# Autodesk Inventor assembly: assembly
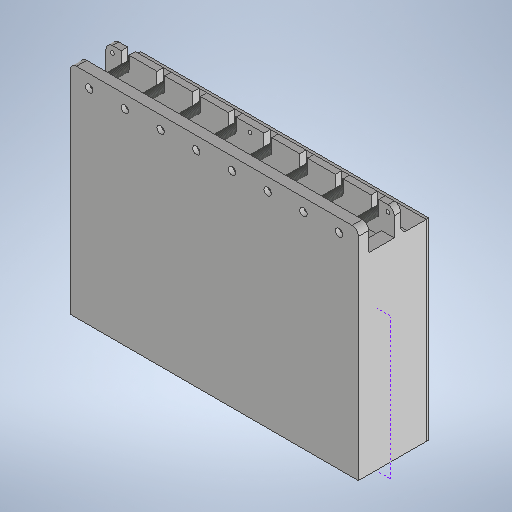
[picture p0: Inventor's stored thumbnail of the model, 512x512]
Saved by Autodesk Inventor 2025.2 (Build 292293000, 293)
## iProperties
Created: 2025-01-01
Part Number: assembly
Document SubType Name: Assembly
Designer: email
Author: email
## Documents named in this file (7)
- C:\Users\email\Desktop\Projects\Capstone\4TB6\CAD_Model\electronics_box\assembly.iam
- C:\Users\email\Desktop\Projects\Capstone\4TB6\CAD_Model\electronics_box\ebox.ipt
- C:\Users\email\Desktop\Projects\Capstone\4TB6\CAD_Model\electronics_box\arduinomega.ipt
- C:\Users\email\Desktop\Projects\Capstone\4TB6\CAD_Model\electronics_box\hx711.ipt
- C:\Users\email\Desktop\Projects\Capstone\4TB6\CAD_Model\electronics_box\motorcontroller.ipt
- C:\Users\email\Documents\Inventor\Content Center Files\R2025\en-US\ISO 7380-1\ISO 7380-1 - M6 x 30.ipt
- C:\Users\email\Desktop\Projects\Capstone\4TB6\CAD_Model\electronics_box\eboxlid.ipt
## Components (13 placed, 6 different names)
1. ebox:1 — Mate:1, Mate:2, Mate:3, Mate:4, Mate:5, Mate:6, Mate:11, Mate:12, Mate:13, Mate:34, Mate:35, Mate:36, Mate:37, Mate:38, Mate:39, Mate:40
2. arduinomega:1 — Mate:1, Mate:2, Mate:3, Mate:4, Mate:5
3. hx711:1 — Mate:11, Mate:12, Mate:13
4. motorcontroller:1 — Mate:6, Mate:34, Mate:35, Mate:36, Mate:37
5. ISO 7380-1 M6 x 30:3
6. ISO 7380-1 M6 x 30:2
7. ISO 7380-1 M6 x 30:4
8. ISO 7380-1 M6 x 30:5
9. ISO 7380-1 M6 x 30:6
10. ISO 7380-1 M6 x 30:7
11. ISO 7380-1 M6 x 30:8
12. ISO 7380-1 M6 x 30:1
13. eboxlid:1 — Mate:38, Mate:39, Mate:40
## Relationships (32: Mate 32)
- Mate:1: ebox:1 ↔ arduinomega:1
- Mate:2: ebox:1 ↔ arduinomega:1
- Mate:3: ebox:1 ↔ arduinomega:1
- Mate:4: ebox:1 ↔ arduinomega:1
- Mate:5: ebox:1 ↔ arduinomega:1
- Mate:6: ebox:1 ↔ motorcontroller:1
- Mate:11: ebox:1 ↔ hx711:1
- Mate:12: ebox:1 ↔ hx711:1
- Mate:13: ebox:1 ↔ hx711:1
- [Mate]: ebox:1 ↔ ISO 7380-1 M6 x 30:2
- [Mate]: ebox:1 ↔ ISO 7380-1 M6 x 30:2
- [Mate]: ebox:1 ↔ ISO 7380-1 M6 x 30:3
- [Mate]: ebox:1 ↔ ISO 7380-1 M6 x 30:3
- [Mate]: ebox:1 ↔ ISO 7380-1 M6 x 30:4
- [Mate]: ebox:1 ↔ ISO 7380-1 M6 x 30:4
- [Mate]: ebox:1 ↔ ISO 7380-1 M6 x 30:5
- [Mate]: ebox:1 ↔ ISO 7380-1 M6 x 30:5
- [Mate]: ebox:1 ↔ ISO 7380-1 M6 x 30:6
- [Mate]: ebox:1 ↔ ISO 7380-1 M6 x 30:6
- [Mate]: ebox:1 ↔ ISO 7380-1 M6 x 30:7
- [Mate]: ebox:1 ↔ ISO 7380-1 M6 x 30:7
- [Mate]: ebox:1 ↔ ISO 7380-1 M6 x 30:8
- [Mate]: ebox:1 ↔ ISO 7380-1 M6 x 30:8
- [Mate]: ebox:1 ↔ ISO 7380-1 M6 x 30:1
- [Mate]: ebox:1 ↔ ISO 7380-1 M6 x 30:1
- Mate:34: ebox:1 ↔ motorcontroller:1
- Mate:35: ebox:1 ↔ motorcontroller:1
- Mate:36: ebox:1 ↔ motorcontroller:1
- Mate:37: ebox:1 ↔ motorcontroller:1
- Mate:38: ebox:1 ↔ eboxlid:1
- Mate:39: ebox:1 ↔ eboxlid:1
- Mate:40: ebox:1 ↔ eboxlid:1
